# Autodesk Inventor assembly: GreyT Telescope Top Block
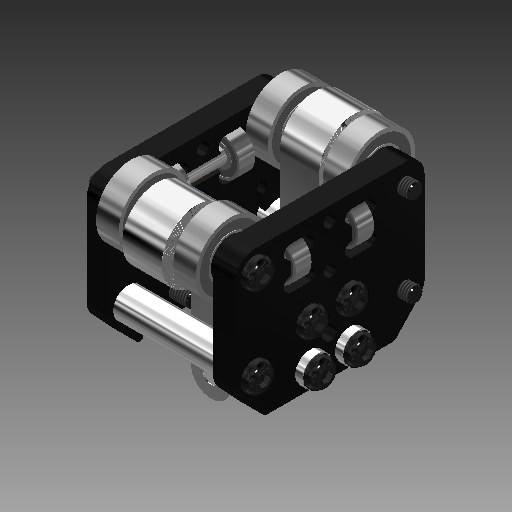
[picture p0: Inventor's stored thumbnail of the model, 512x512]
Saved by Autodesk Inventor 2023 (Build 270158000, 158)
## iProperties
Created: 2021-12-31
Part Number: GreyT Telescope Top Block
Document SubType Name: Assembly
Mass: 297.481 g
Surface Area: 483.09 cm^2
Volume: 62.0606 cm^3
Density: 4.7934 g/cm^3
Revision Number: ANY
## Documents named in this file (16)
- E:\Collaborative Robots\Collaborative Part Library\Elevators\GreyT Telescope\1.5 in Top Block WCP-0418.iam
- E:\Collaborative Robots\Collaborative Part Library\Elevators\GreyT Telescope\Smallest Stage\WCP-0418-003 Rev1.ipt
- E:\Collaborative Robots\Collaborative Part Library\Elevators\GreyT Telescope\WCP-0418-005 Rev1.ipt
- E:\Collaborative Robots\Collaborative Part Library\Power Transfer\Bearings and Bushings\Bearings\R6.ipt
- C:\Users\Cal\Desktop\Robotics\Design\Collaborative\Collaborative Parts Library\Power Transfer\Bearings and Bushings\Bearings.ipt
- E:\Collaborative Robots\Collaborative Part Library\Power Transfer\Bearings and Bushings\Bearings\R3ZZ.ipt
- E:\Collaborative Robots\Collaborative Part Library\Hardware\Dowel Pins\Dowel Pins\0.1875in  x 1.25in Stainless Steel Dowel Pin.ipt
- C:\Users\Cal\Desktop\Robotics\Design\Collaborative\Collaborative Parts Library\Hardware\Dowel Pins\Dowel Pins.ipt
- E:\Collaborative Robots\Collaborative Part Library\Hardware\Fasteners\Machine Screws\10-32 UNFx0.375 Button Head Cap Screw.ipt
- C:\Users\Cal\Desktop\Robotics\Design\Collaborative\Collaborative Parts Library\Hardware\Fasteners\Machine Screws.ipt
- E:\Collaborative Robots\Collaborative Part Library\Hardware\Spacers\Spacers & Standoffs\Aluminum Unthreaded Spacer (No. 10 x 0.094Lg x 0.375OD).ipt
- C:\Users\Cal\Desktop\Robotics\Design\Collaborative\Collaborative Parts Library\Hardware\Spacers\Spacers & Standoffs.ipt
- E:\Collaborative Robots\Collaborative Part Library\Hardware\Fasteners\Machine Screws\10-32 UNFx0.5 Button Head Cap Screw.ipt
- E:\Collaborative Robots\Collaborative Part Library\Hardware\Fasteners\Machine Screws\10-32 UNFx2 Button Head Cap Screw.ipt
- E:\Collaborative Robots\Collaborative Part Library\Hardware\Spacers\Spacers & Standoffs\Aluminum Unthreaded Spacer (No. 10 x 1.5Lg x 0.375OD).ipt
- E:\Collaborative Robots\Collaborative Part Library\Elevators\GreyT Telescope\GreyT Constant Force Spring.ipt
## Components (36 placed, 11 different names)
1. Aluminum Unthreaded Spacer (No. 10 x 1.5Lg x 0.375OD):5 — Insert:22, Mate:8
2. Aluminum Unthreaded Spacer (No. 10 x 1.5Lg x 0.375OD):6 — Insert:21, Insert:25, Symmetry:4
3. Aluminum Unthreaded Spacer (No. 10 x 1.5Lg x 0.375OD):7 — Insert:24, Mate:7
4. Aluminum Unthreaded Spacer (No. 10 x 1.5Lg x 0.375OD):8 — Insert:23, Symmetry:4
5. WCP-0418-003 Rev1:1 — Insert:1, Insert:2, Insert:5, Insert:6, Insert:9, Insert:10, Insert:17, Insert:18, Tangent:1, Tangent:4, Mate:5, Insert:24, Insert:25, Symmetry:3, Mate:6
6. WCP-0418-003 Rev1:2 — Insert:3, Insert:4, Insert:7, Insert:8, Insert:11, Insert:12, Insert:19, Insert:20, Tangent:2, Tangent:3, Insert:21, Insert:22, Insert:23, Symmetry:3
7. 10-32 UNFx2 Button Head Cap Screw:9 — Insert:17
8. 10-32 UNFx2 Button Head Cap Screw:10 — Insert:18
9. 10-32 UNFx2 Button Head Cap Screw:11 — Insert:19
10. 10-32 UNFx2 Button Head Cap Screw:12 — Insert:20
11. 10-32 UNFx0.375 Button Head Cap Screw:1 — Insert:5
12. 10-32 UNFx0.375 Button Head Cap Screw:2 — Insert:6
13. 10-32 UNFx0.5 Button Head Cap Screw:5 — Insert:14
14. 10-32 UNFx0.5 Button Head Cap Screw:6 — Insert:13
15. 10-32 UNFx0.5 Button Head Cap Screw:7 — Insert:15
16. 10-32 UNFx0.5 Button Head Cap Screw:8 — Insert:16
17. 10-32 UNFx0.375 Button Head Cap Screw:3 — Insert:7
18. 10-32 UNFx0.375 Button Head Cap Screw:4 — Insert:8
19. 0.1875in  x 1.25in Stainless Steel Dowel Pin:1 — Mate:2, Flush:3, Tangent:1, Tangent:4
20. 0.1875in  x 1.25in Stainless Steel Dowel Pin:2 — Mate:4, Flush:3, Tangent:2, Tangent:3
21. R3ZZ:5 — Mate:1, Mate:2, Flush:1, Symmetry:1, Symmetry:2, Mate:5
22. R3ZZ:6 — Mate:1, Flush:2, Symmetry:1, Symmetry:2
23. R3ZZ:7 — Mate:3, Mate:4, Flush:1
24. R3ZZ:8 — Mate:3, Flush:2
25. R6:1 — Insert:4, Symmetry:5
26. R6:2 — Insert:2, Symmetry:5
27. R6:3 — Insert:1
28. R6:4 — Insert:3
29. WCP-0418-005 Rev1:1 — Flush:6, Mate:8, Flush:7, Tangent:8
30. WCP-0418-005 Rev1:2 — Tangent:7, Flush:6, Mate:7
31. Aluminum Unthreaded Spacer (No. 10 x 0.094Lg x 0.375OD):1 — Insert:9, Insert:13
32. Aluminum Unthreaded Spacer (No. 10 x 0.094Lg x 0.375OD):2 — Insert:11, Insert:15
33. Aluminum Unthreaded Spacer (No. 10 x 0.094Lg x 0.375OD):3 — Insert:12, Insert:16
34. Aluminum Unthreaded Spacer (No. 10 x 0.094Lg x 0.375OD):4 — Insert:10, Insert:14
35. GreyT Constant Force Spring:1 — Symmetry:6, Symmetry:7, Flush:5, Flush:8, Tangent:8, Mate:9
36. GreyT Constant Force Spring:2 — Symmetry:6, Symmetry:7, Flush:5, Tangent:7, Flush:8, Mate:9
## Relationships (54: Insert 25, Mate 9, Flush 7, Symmetry 7, Tangent 6)
- Insert:1: WCP-0418-003 Rev1:1 ↔ R6:3
- Insert:2: WCP-0418-003 Rev1:1 ↔ R6:2
- Insert:3: WCP-0418-003 Rev1:2 ↔ R6:4
- Insert:4: WCP-0418-003 Rev1:2 ↔ R6:1
- Mate:1: R3ZZ:5 ↔ R3ZZ:6
- Mate:2: 0.1875in  x 1.25in Stainless Steel Dowel Pin:1 ↔ R3ZZ:5
- Mate:3: R3ZZ:7 ↔ R3ZZ:8
- Mate:4: 0.1875in  x 1.25in Stainless Steel Dowel Pin:2 ↔ R3ZZ:7
- Flush:1: R3ZZ:5 ↔ R3ZZ:7
- Flush:2: R3ZZ:6 ↔ R3ZZ:8
- Symmetry:1: R3ZZ:5 ↔ R3ZZ:6
- Flush:3: 0.1875in  x 1.25in Stainless Steel Dowel Pin:1 ↔ 0.1875in  x 1.25in Stainless Steel Dowel Pin:2
- Symmetry:2: R3ZZ:5 ↔ R3ZZ:6
- Insert:5: WCP-0418-003 Rev1:1 ↔ 10-32 UNFx0.375 Button Head Cap Screw:1
- Insert:6: WCP-0418-003 Rev1:1 ↔ 10-32 UNFx0.375 Button Head Cap Screw:2
- Insert:7: WCP-0418-003 Rev1:2 ↔ 10-32 UNFx0.375 Button Head Cap Screw:3
- Insert:8: WCP-0418-003 Rev1:2 ↔ 10-32 UNFx0.375 Button Head Cap Screw:4
- Insert:9: WCP-0418-003 Rev1:1 ↔ Aluminum Unthreaded Spacer (No. 10 x 0.094Lg x 0.375OD):1
- Insert:10: WCP-0418-003 Rev1:1 ↔ Aluminum Unthreaded Spacer (No. 10 x 0.094Lg x 0.375OD):4
- Insert:11: WCP-0418-003 Rev1:2 ↔ Aluminum Unthreaded Spacer (No. 10 x 0.094Lg x 0.375OD):2
- Insert:12: WCP-0418-003 Rev1:2 ↔ Aluminum Unthreaded Spacer (No. 10 x 0.094Lg x 0.375OD):3
- Insert:13: 10-32 UNFx0.5 Button Head Cap Screw:6 ↔ Aluminum Unthreaded Spacer (No. 10 x 0.094Lg x 0.375OD):1
- Insert:14: 10-32 UNFx0.5 Button Head Cap Screw:5 ↔ Aluminum Unthreaded Spacer (No. 10 x 0.094Lg x 0.375OD):4
- Insert:15: 10-32 UNFx0.5 Button Head Cap Screw:7 ↔ Aluminum Unthreaded Spacer (No. 10 x 0.094Lg x 0.375OD):2
- Insert:16: 10-32 UNFx0.5 Button Head Cap Screw:8 ↔ Aluminum Unthreaded Spacer (No. 10 x 0.094Lg x 0.375OD):3
- Insert:17: WCP-0418-003 Rev1:1 ↔ 10-32 UNFx2 Button Head Cap Screw:9
- Insert:18: WCP-0418-003 Rev1:1 ↔ 10-32 UNFx2 Button Head Cap Screw:10
- Insert:19: WCP-0418-003 Rev1:2 ↔ 10-32 UNFx2 Button Head Cap Screw:11
- Insert:20: WCP-0418-003 Rev1:2 ↔ 10-32 UNFx2 Button Head Cap Screw:12
- Tangent:1: WCP-0418-003 Rev1:1 ↔ 0.1875in  x 1.25in Stainless Steel Dowel Pin:1
- Tangent:2: WCP-0418-003 Rev1:2 ↔ 0.1875in  x 1.25in Stainless Steel Dowel Pin:2
- Tangent:3: WCP-0418-003 Rev1:2 ↔ 0.1875in  x 1.25in Stainless Steel Dowel Pin:2
- Tangent:4: WCP-0418-003 Rev1:1 ↔ 0.1875in  x 1.25in Stainless Steel Dowel Pin:1
- Mate:5: WCP-0418-003 Rev1:1 ↔ R3ZZ:5
- Insert:21: Aluminum Unthreaded Spacer (No. 10 x 1.5Lg x 0.375OD):6 ↔ WCP-0418-003 Rev1:2
- Insert:22: Aluminum Unthreaded Spacer (No. 10 x 1.5Lg x 0.375OD):5 ↔ WCP-0418-003 Rev1:2
- Insert:23: Aluminum Unthreaded Spacer (No. 10 x 1.5Lg x 0.375OD):8 ↔ WCP-0418-003 Rev1:2
- Insert:24: Aluminum Unthreaded Spacer (No. 10 x 1.5Lg x 0.375OD):7 ↔ WCP-0418-003 Rev1:1
- Insert:25: Aluminum Unthreaded Spacer (No. 10 x 1.5Lg x 0.375OD):6 ↔ WCP-0418-003 Rev1:1
- Symmetry:3: WCP-0418-003 Rev1:1 ↔ WCP-0418-003 Rev1:2
- Symmetry:4: Aluminum Unthreaded Spacer (No. 10 x 1.5Lg x 0.375OD):6 ↔ Aluminum Unthreaded Spacer (No. 10 x 1.5Lg x 0.375OD):8
- Mate:6: WCP-0418-003 Rev1:1
- Symmetry:5: R6:1 ↔ R6:2
- Symmetry:6: GreyT Constant Force Spring:1 ↔ GreyT Constant Force Spring:2
- Symmetry:7: GreyT Constant Force Spring:1 ↔ GreyT Constant Force Spring:2
- Flush:5: GreyT Constant Force Spring:1 ↔ GreyT Constant Force Spring:2
- Tangent:7: WCP-0418-005 Rev1:2 ↔ GreyT Constant Force Spring:2
- Flush:6: WCP-0418-005 Rev1:1 ↔ WCP-0418-005 Rev1:2
- Mate:7: Aluminum Unthreaded Spacer (No. 10 x 1.5Lg x 0.375OD):7 ↔ WCP-0418-005 Rev1:2
- Mate:8: Aluminum Unthreaded Spacer (No. 10 x 1.5Lg x 0.375OD):5 ↔ WCP-0418-005 Rev1:1
- Flush:7: WCP-0418-005 Rev1:1
- Flush:8: GreyT Constant Force Spring:1 ↔ GreyT Constant Force Spring:2
- Tangent:8: WCP-0418-005 Rev1:1 ↔ GreyT Constant Force Spring:1
- Mate:9: GreyT Constant Force Spring:1 ↔ GreyT Constant Force Spring:2
